# Autodesk Inventor assembly: 20-058-PHTM-HRDSET-01
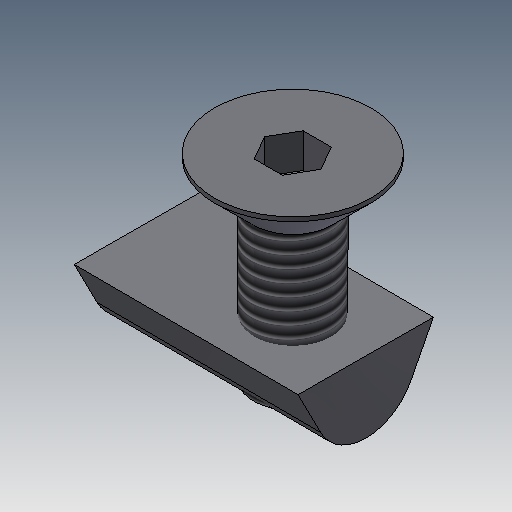
[picture p0: Inventor's stored thumbnail of the model, 512x512]
Saved by Autodesk Inventor 2018.3 (Build 223284000, 284)
## iProperties
Created: 2004-11-17
Part Number: 20-058-PHTM-HRDSET-01
Document SubType Name: Assembly
Designer: Autodesk, Inc.
Manufacturer: Standard
Standards Organization: Custom
Description: MISC HADWARE SET PHANTOM
Catalog Web Link: http://www.parker.com/ead/cm1.asp?cmid=809
Vendor: PARKER IPS
Mass: 20.6187 g
Surface Area: 19.5863 cm^2
Volume: 2.62994 cm^3
Density: 7.84 g/cm^3
CAGE: 1LJX3
Dept. ID: Product Design
Description #2: ---
Finish #1: ---
Finish #2: ---
Material ID: ---
Project Number: ---
Author: Autodesk, Inc.
## Documents named in this file (5)
- C:\AVAInvAPI\Workspace\Test Station\Components\M178-1000-Phantom01.iam
- C:\AVAInvAPI\Workspace\Test Station\Components\24-220-8.ipt
- C:\AVAInvAPI\Workspace\Test Station\Components\20-058.ipt
- C:\Users\kelleyb.ADS\Desktop\Samples MIGRATED 2009 224 RTM_1\Standard Parts\Test Station Content\Fastners\2X-YYY-ZZ IPS Screws.ipt
- C:\Users\kelleyb.ADS\Desktop\Samples MIGRATED 2009 224 RTM_1\Standard Parts\Test Station Content\Fastners\20-XXX TSlot Nuts.ipt
## Components (2 placed, 2 different names)
1. 24-220-8:1
2. 20-058:1
## Relationships (1: Insert 1)
- [Insert] (-14.224 mm): 24-220-8:1 ↔ 20-058:1
